# Autodesk Inventor assembly: ASSY_TREBUCHET_DESIGN2
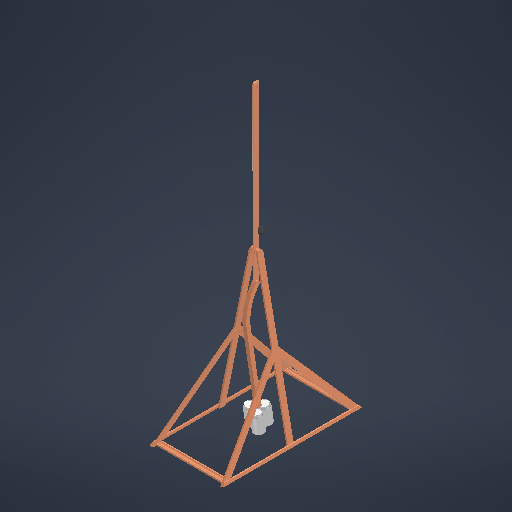
[picture p0: Inventor's stored thumbnail of the model, 512x512]
Saved by Autodesk Inventor 2026.2 (Build 302298010, 298A)
## iProperties
Created: 2026-02-10
Part Number: ASSY_TREBUCHET_DESIGN2
Document SubType Name: Assembly
Designer: 4aida
Mass: 2977.99 g
Surface Area: 11813.1 cm^2
Volume: 3545.13 cm^3
Density: 0.840022 g/cm^3
Author: 4aida
## Documents named in this file (10)
- C:\Users\4aida\OneDrive\Documents\GitHub\Design_II_Group6\Trebuchet\WIPPER_TREBUCHET\ASSY_TREBUCHET_DESIGN2.iam
- C:\Users\4aida\OneDrive\Documents\GitHub\Design_II_Group6\Trebuchet\Canette-355ml.ipt
- C:\Users\4aida\OneDrive\Documents\GitHub\Design_II_Group6\Trebuchet\Yellow_dot_squash_ball,Trebuchet.ipt
- C:\Users\4aida\OneDrive\Documents\GitHub\Design_II_Group6\Trebuchet\WIPPER_TREBUCHET\wipper_arm.ipt
- C:\Users\4aida\OneDrive\Documents\GitHub\Design_II_Group6\Trebuchet\COUNTERWEIGHT_OUTSIDE_ARM,TREBUCHET.ipt
- C:\Users\4aida\OneDrive\Documents\GitHub\Design_II_Group6\Trebuchet\PIVOT_SPACERS,TREBUCHET.ipt
- C:\Users\4aida\OneDrive\Documents\GitHub\Design_II_Group6\Trebuchet\WIPPER_TREBUCHET\BASE_FRONT,BACK_TREBUCHET.ipt
- C:\Users\4aida\OneDrive\Documents\GitHub\Design_II_Group6\Trebuchet\WIPPER_TREBUCHET\BASE_SIDEK_TREBUCHET.ipt
- C:\Users\4aida\OneDrive\Documents\GitHub\Design_II_Group6\Trebuchet\WIPPER_TREBUCHET\UPRIGHTS_TREBUCHET.ipt
- C:\Users\4aida\OneDrive\Documents\GitHub\Design_II_Group6\Trebuchet\WIPPER_TREBUCHET\SUPPORTS_TREBUCHET.ipt
## Components (18 placed, 9 different names)
1. Canette-355ml:1 — Tangent:1, Tangent:2, Flush:1, Flush:2, Mate:57
2. Yellow_dot_squash_ball,Trebuchet:1 — Mate:45
3. Canette-355ml:2 — Tangent:2, Tangent:3, Flush:2
4. Canette-355ml:3 — Tangent:1, Tangent:3, Flush:1
5. BASE_FRONT,BACK_TREBUCHET:1 — Flush:40, Flush:42
6. BASE_FRONT,BACK_TREBUCHET:3 — Flush:28, Flush:41, Flush:42
7. UPRIGHTS_TREBUCHET:1 — Mate:38, Flush:29, Flush:30, Mate:48, Mate:49, Mate:50, Mate:51, Mate:52, Flush:39, Flush:41
8. UPRIGHTS_TREBUCHET:2 — Flush:31, Flush:32, Mate:46, Mate:47, Mate:50, Mate:53, Mate:54, Flush:39, Angle:1, Flush:40
9. PIVOT_SPACERS,TREBUCHET:3 — Mate:40, Mate:41
10. PIVOT_SPACERS,TREBUCHET:4 — Mate:42, Mate:43
11. wipper_arm:3 — Mate:39, Mate:40, Mate:41, Mate:42, Mate:43, Mate:44, Mate:45, Mate:55, Mate:56
12. SUPPORTS_TREBUCHET:1 — Flush:30, Mate:49, Flush:33, Flush:35
13. SUPPORTS_TREBUCHET:2 — Flush:32, Mate:46, Flush:37, Flush:38
14. SUPPORTS_TREBUCHET:3 — Flush:29, Mate:48, Flush:34
15. SUPPORTS_TREBUCHET:4 — Flush:31, Mate:47, Flush:36
16. BASE_SIDEK_TREBUCHET:3 — Mate:51, Flush:33, Flush:34, Mate:52, Flush:35
17. BASE_SIDEK_TREBUCHET:4 — Mate:53, Flush:36, Flush:37, Flush:38, Mate:54
18. COUNTERWEIGHT_OUTSIDE_ARM,TREBUCHET:3 — Mate:55, Mate:56, Mate:57
## Relationships (41: Mate 20, Flush 17, Tangent 3, Angle 1)
- Tangent:1: Canette-355ml:1 ↔ Canette-355ml:3
- Tangent:2: Canette-355ml:1 ↔ Canette-355ml:2
- Tangent:3: Canette-355ml:2 ↔ Canette-355ml:3
- Flush:1: Canette-355ml:1 ↔ Canette-355ml:3
- Flush:2: Canette-355ml:1 ↔ Canette-355ml:2
- Flush:28: BASE_FRONT,BACK_TREBUCHET:3
- Mate:38: UPRIGHTS_TREBUCHET:1
- Mate:39: wipper_arm:3
- Mate:40: PIVOT_SPACERS,TREBUCHET:3 ↔ wipper_arm:3
- Mate:41: PIVOT_SPACERS,TREBUCHET:3 ↔ wipper_arm:3
- Mate:42: PIVOT_SPACERS,TREBUCHET:4 ↔ wipper_arm:3
- Mate:43: PIVOT_SPACERS,TREBUCHET:4 ↔ wipper_arm:3
- Mate:44: wipper_arm:3
- Mate:45: Yellow_dot_squash_ball,Trebuchet:1 ↔ wipper_arm:3
- Flush:29: UPRIGHTS_TREBUCHET:1 ↔ SUPPORTS_TREBUCHET:3
- Flush:30: UPRIGHTS_TREBUCHET:1 ↔ SUPPORTS_TREBUCHET:1
- Flush:31: UPRIGHTS_TREBUCHET:2 ↔ SUPPORTS_TREBUCHET:4
- Flush:32: UPRIGHTS_TREBUCHET:2 ↔ SUPPORTS_TREBUCHET:2
- Mate:46: UPRIGHTS_TREBUCHET:2 ↔ SUPPORTS_TREBUCHET:2
- Mate:47: UPRIGHTS_TREBUCHET:2 ↔ SUPPORTS_TREBUCHET:4
- Mate:48: UPRIGHTS_TREBUCHET:1 ↔ SUPPORTS_TREBUCHET:3
- Mate:49: UPRIGHTS_TREBUCHET:1 ↔ SUPPORTS_TREBUCHET:1
- Mate:50: UPRIGHTS_TREBUCHET:1 ↔ UPRIGHTS_TREBUCHET:2
- Mate:51: UPRIGHTS_TREBUCHET:1 ↔ BASE_SIDEK_TREBUCHET:3
- Flush:33: SUPPORTS_TREBUCHET:1 ↔ BASE_SIDEK_TREBUCHET:3
- Flush:34: SUPPORTS_TREBUCHET:3 ↔ BASE_SIDEK_TREBUCHET:3
- Mate:52: UPRIGHTS_TREBUCHET:1 ↔ BASE_SIDEK_TREBUCHET:3
- Flush:35: SUPPORTS_TREBUCHET:1 ↔ BASE_SIDEK_TREBUCHET:3
- Mate:53: UPRIGHTS_TREBUCHET:2 ↔ BASE_SIDEK_TREBUCHET:4
- Flush:36: SUPPORTS_TREBUCHET:4 ↔ BASE_SIDEK_TREBUCHET:4
- Flush:37: SUPPORTS_TREBUCHET:2 ↔ BASE_SIDEK_TREBUCHET:4
- Flush:38: SUPPORTS_TREBUCHET:2 ↔ BASE_SIDEK_TREBUCHET:4
- Mate:54: UPRIGHTS_TREBUCHET:2 ↔ BASE_SIDEK_TREBUCHET:4
- Flush:39: UPRIGHTS_TREBUCHET:1 ↔ UPRIGHTS_TREBUCHET:2
- Angle:1 (180 deg): UPRIGHTS_TREBUCHET:2
- Flush:40: BASE_FRONT,BACK_TREBUCHET:1 ↔ UPRIGHTS_TREBUCHET:2
- Mate:55: wipper_arm:3 ↔ COUNTERWEIGHT_OUTSIDE_ARM,TREBUCHET:3
- Mate:56: wipper_arm:3 ↔ COUNTERWEIGHT_OUTSIDE_ARM,TREBUCHET:3
- Mate:57: Canette-355ml:1 ↔ COUNTERWEIGHT_OUTSIDE_ARM,TREBUCHET:3
- Flush:41: BASE_FRONT,BACK_TREBUCHET:3 ↔ UPRIGHTS_TREBUCHET:1
- Flush:42: BASE_FRONT,BACK_TREBUCHET:1 ↔ BASE_FRONT,BACK_TREBUCHET:3
